# Autodesk Inventor assembly: QuadCopter
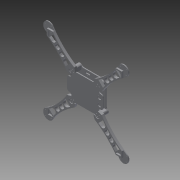
[picture p0: Inventor's stored thumbnail of the model, 180x180]
Saved by Autodesk Inventor 2015 (Build 190159000, 159)
## iProperties
Created: 2015-06-01
Part Number: QuadCopter
Document SubType Name: Assembly
Designer: Vu
Author: Vu
## Documents named in this file (4)
- C:\Users\Vu\Documents\QuadCopter\models\heavyRevision\QuadCopter.iam
- C:\Users\Vu\Documents\QuadCopter\models\heavyRevision\LowerPlatter.ipt
- C:\Users\Vu\Documents\QuadCopter\models\heavyRevision\Arm.ipt
- C:\Users\Vu\Documents\QuadCopter\models\heavyRevision\Ceiling.ipt
## Components (6 placed, 3 different names)
1. LowerPlatter:1 — Mate:1, Mate:2, Mate:3, Mate:4, Mate:5, Mate:6, Mate:7, Mate:8, Mate:9, Mate:10, Mate:11, Mate:12
2. Arm:1 — Mate:1, Mate:2, Mate:3, Mate:13
3. Arm:2 — Mate:4, Mate:5, Mate:6
4. Arm:3 — Mate:10, Mate:11, Mate:12
5. Arm:4 — Mate:7, Mate:8, Mate:9, Mate:14, Mate:15
6. Ceiling:1 — Mate:13, Mate:14, Mate:15
## Relationships (15: Mate 15)
- Mate:1: LowerPlatter:1 ↔ Arm:1
- Mate:2: LowerPlatter:1 ↔ Arm:1
- Mate:3: LowerPlatter:1 ↔ Arm:1
- Mate:4: LowerPlatter:1 ↔ Arm:2
- Mate:5: LowerPlatter:1 ↔ Arm:2
- Mate:6: LowerPlatter:1 ↔ Arm:2
- Mate:7: LowerPlatter:1 ↔ Arm:4
- Mate:8: LowerPlatter:1 ↔ Arm:4
- Mate:9: LowerPlatter:1 ↔ Arm:4
- Mate:10: LowerPlatter:1 ↔ Arm:3
- Mate:11: LowerPlatter:1 ↔ Arm:3
- Mate:12: LowerPlatter:1 ↔ Arm:3
- Mate:13: Arm:1 ↔ Ceiling:1
- Mate:14: Arm:4 ↔ Ceiling:1
- Mate:15: Arm:4 ↔ Ceiling:1
